# Autodesk Inventor assembly: asmTemp
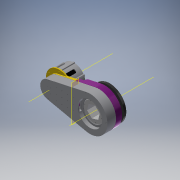
[picture p0: Inventor's stored thumbnail of the model, 180x180]
Saved by Autodesk Inventor 2018 (Build 220112000, 112)
## iProperties
Created: 2019-11-13
Part Number: asmTemp
Document SubType Name: Assembly
Designer: Bunny320
Author: Bunny320
## Documents named in this file (11)
- C:\Users\Bunny320\Desktop\sechs\4-CAD\10-J1.iam
- C:\Users\Bunny320\Desktop\sechs\4-CAD\101-bottom.ipt
- C:\Users\Bunny320\Desktop\sechs\4-CAD\generated\J1_belt.iam
- C:\Users\Bunny320\Desktop\sechs\4-CAD\standardParts\61814-2RS1\61814-2RS1.iam
- C:\Users\Bunny320\Desktop\sechs\4-CAD\AS5047.ipt
- C:\Users\Bunny320\Desktop\sechs\4-CAD\magnet-6x2.5.ipt
- C:\Users\Bunny320\Desktop\sechs\4-CAD\103-top-output.ipt
- C:\Users\Bunny320\Desktop\sechs\4-CAD\standardParts\SUNNYSKY-X6215S-kv170\X6215S.ipt
- C:\Users\Bunny320\Desktop\sechs\4-CAD\104-motor-case-new.ipt
- C:\Users\Bunny320\Desktop\sechs\4-CAD\102-top-motor-adapt-big-motor.ipt
- C:\Users\Bunny320\Desktop\sechs\4-CAD\105-flange adapter.ipt
## Components (11 placed, 10 different names)
1. 101-bottom:1 — Flush:1, Flush:2, Flush:3, Mate:5, Mate:17, Mate:18, Mate:28
2. J1_belt:1 [sub-assembly] — Mate:1, Mate:2, Mate:3, Mate:6, Mate:7, Mate:8, Mate:9, Mate:10, Mate:20, Mate:26, Mate:27, Mate:30, Mate:31
3. 61814-2RS1:1 [sub-assembly] — Mate:2, Mate:8
4. 61814-2RS1:2 [sub-assembly] — Mate:3, Mate:5, Mate:7
5. AS5047:1 — Mate:21, Mate:22, Mate:23
6. magnet-6x2.5:1 — Mate:9, Mate:10
7. 103-top-output:1 — Mate:17, Mate:18
8. X6215S:1 — Mate:24, Mate:25, Mate:26
9. 104-motor-case-new:1 — Mate:20, Mate:21, Mate:22, Mate:23, Mate:24, Mate:25
10. 102-top-motor-adapt-big-motor:1 — Mate:27, Mate:28, Mate:29
11. 105-flange adapter:1 — Mate:30, Mate:31
## Relationships (26: Mate 23, Flush 3)
- Flush:1: 101-bottom:1
- Flush:2: 101-bottom:1
- Flush:3: 101-bottom:1
- Mate:1: J1_belt:1
- Mate:2: J1_belt:1 ↔ 61814-2RS1:1
- Mate:3: J1_belt:1 ↔ 61814-2RS1:2
- Mate:5: 101-bottom:1 ↔ 61814-2RS1:2
- Mate:6: J1_belt:1
- Mate:7: J1_belt:1 ↔ 61814-2RS1:2
- Mate:8: J1_belt:1 ↔ 61814-2RS1:1
- Mate:9: J1_belt:1 ↔ magnet-6x2.5:1
- Mate:10: J1_belt:1 ↔ magnet-6x2.5:1
- Mate:17: 101-bottom:1 ↔ 103-top-output:1
- Mate:18: 101-bottom:1 ↔ 103-top-output:1
- Mate:20: J1_belt:1 ↔ 104-motor-case-new:1
- Mate:21: AS5047:1 ↔ 104-motor-case-new:1
- Mate:22: AS5047:1 ↔ 104-motor-case-new:1
- Mate:23: AS5047:1 ↔ 104-motor-case-new:1
- Mate:24: X6215S:1 ↔ 104-motor-case-new:1
- Mate:25: X6215S:1 ↔ 104-motor-case-new:1
- Mate:26: J1_belt:1 ↔ X6215S:1
- Mate:27: J1_belt:1 ↔ 102-top-motor-adapt-big-motor:1
- Mate:28: 101-bottom:1 ↔ 102-top-motor-adapt-big-motor:1
- Mate:29: 102-top-motor-adapt-big-motor:1
- Mate:30: J1_belt:1 ↔ 105-flange adapter:1
- Mate:31: J1_belt:1 ↔ 105-flange adapter:1
